# Autodesk Inventor assembly: 2AM-17-A-2200 - slider outside
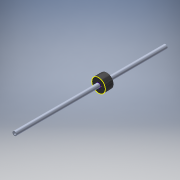
[picture p0: Inventor's stored thumbnail of the model, 180x180]
Saved by Autodesk Inventor 2017 (Build 210142000, 142)
## iProperties
Created: 2017-12-27
Part Number: 2AM-17-A-2200 - slider outside
Document SubType Name: Assembly
Designer: Micah
Author: Micah
## Documents named in this file (4)
- C:\Users\Micah\Desktop\inventor\CADathon-2017\2AM-17-A-0200 - Smokestack Elevator\2AM-17-A-2200 - slider outside.iam
- C:\Users\Micah\Desktop\inventor\CADathon-2017\2AM-17-A-0200 - Smokestack Elevator\COTS\2in Wheel Intergrated 0500 HEX Hub.ipt
- C:\Users\Micah\Desktop\inventor\CADathon-2017\2AM-17-A-0200 - Smokestack Elevator\COTS\1_2_OD_Tube_Axle_Stock_18_217-3311.ipt
- C:\Users\Micah\Desktop\inventor\CADathon-2017\2AM-17-A-0200 - Smokestack Elevator\2AM-17-P-1202 - hex to tube adapter.ipt
## Components (3 placed, 3 different names)
1. 2in Wheel Intergrated 0500 HEX Hub:1 — Rigid:1
2. 1_2_OD_Tube_Axle_Stock_18_217-3311:1 — Rotational:1
3. 2AM-17-P-1202 - hex to tube adapter:1 — Rigid:1, Rotational:1
## Relationships (2: WeldJoint 1, RevoluteJoint 1)
- Rigid:1 [WeldJoint]: 2in Wheel Intergrated 0500 HEX Hub:1 ↔ 2AM-17-P-1202 - hex to tube adapter:1
- Rotational:1 [RevoluteJoint] (-177.8 mm): 1_2_OD_Tube_Axle_Stock_18_217-3311:1 ↔ 2AM-17-P-1202 - hex to tube adapter:1
